# Autodesk Inventor assembly: s-assy-tentioner
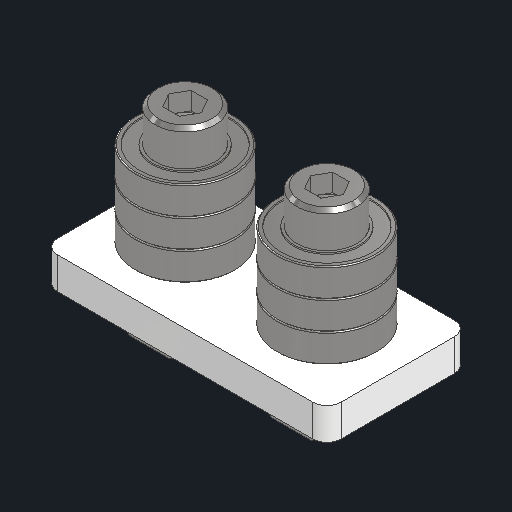
[picture p0: Inventor's stored thumbnail of the model, 512x512]
Saved by Autodesk Inventor 2022 (Build 260153000, 153)
## iProperties
Created: 2021-10-17
Part Number: s-assy-tentioner
Document SubType Name: Assembly
Designer: Yuta Kage
Author: Yuta Kage
## Documents named in this file (5)
- C:\Users\yuta0\Documents\GitHub\catchrobo_hardware\assy-scara\s-assy-tentioner.iam
- C:\Users\yuta0\Documents\GitHub\catchrobo_hardware\assy-scara\scara-base4.ipt
- C:\Users\yuta0\Documents\GitHub\catchrobo_hardware\assy-scara\MR148ZZ.ipt
- C:\Users\yuta0\Documents\GitHub\catchrobo_hardware\assy-scara\HNTT5-5.ipt
- C:\Users\yuta0\Documents\GitHub\catchrobo_hardware\assy-scara\CB5-22.ipt
## Components (11 placed, 4 different names)
1. scara-base4:1 — メイト:1, メイト:2, メイト:5, 角度:1, メイト:6, メイト:7, メイト:8
2. MR148ZZ:1 — メイト:1, メイト:2
3. MR148ZZ:2
4. MR148ZZ:3
5. MR148ZZ:4
6. MR148ZZ:5
7. MR148ZZ:6
8. HNTT5-5:1 — メイト:5, 角度:1, メイト:6
9. CB5-22:1 — メイト:7, メイト:8
10. HNTT5-5:2
11. CB5-22:2
## Component patterns: (6 elements, first: MR148ZZ:1), (2 elements, first: HNTT5-5:1 + CB5-22:1)
## Relationships (7: Mate 6, Angle 1)
- メイト:1 [Mate]: scara-base4:1 ↔ MR148ZZ:1
- メイト:2 [Mate]: scara-base4:1 ↔ MR148ZZ:1
- メイト:5 [Mate]: scara-base4:1 ↔ HNTT5-5:1
- 角度:1 [Angle] (0 deg): scara-base4:1 ↔ HNTT5-5:1
- メイト:6 [Mate] (2 mm): scara-base4:1 ↔ HNTT5-5:1
- メイト:7 [Mate]: scara-base4:1 ↔ CB5-22:1
- メイト:8 [Mate]: scara-base4:1 ↔ CB5-22:1
